# Autodesk Inventor assembly: Trilho 60 min - 12 horas montado
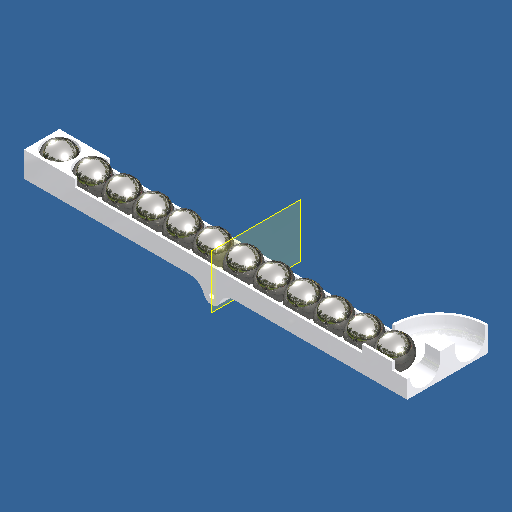
[picture p0: Inventor's stored thumbnail of the model, 512x512]
Saved by Autodesk Inventor 2024 (Build 280153000, 153)
## iProperties
Created: 2023-05-16
Part Number: Trilho 60 min - 12 horas montado
Document SubType Name: Assembly
Designer: jpjoa
Mass: 338.261 g
Surface Area: 330.699 cm^2
Volume: 65.9182 cm^3
Density: 5.13152 g/cm^3
Author: jpjoa
## Documents named in this file (3)
- G:\.shortcut-targets-by-id\16j0rtmAzHYi4Hd3siOhaEHA2SaTRFf-m\Marbles - Peças novas\Trilho 60 min - 12 horas montado.iam
- G:\.shortcut-targets-by-id\16j0rtmAzHYi4Hd3siOhaEHA2SaTRFf-m\Marbles - Peças novas\Trilho 60 min - 12 horas.ipt
- G:\.shortcut-targets-by-id\16j0rtmAzHYi4Hd3siOhaEHA2SaTRFf-m\Marbles - Peças novas\Bola.ipt
## Components (13 placed, 2 different names)
1. Trilho 60 min - 12 horas:1 — Coincidente:1, Coincidente:2, Coincidente:3, Coincidente:4, Coincidente:5, Coincidente:6, Coincidente:7, Coincidente:8, Coincidente:9, Coincidente:10, Coincidente:11, Coincidente:12
2. Bola:1 — Coincidente:1
3. Bola:2 — Coincidente:2, Tangente:1
4. Bola:3 — Coincidente:3, Tangente:1, Tangente:2
5. Bola:4 — Coincidente:4, Tangente:2, Tangente:3
6. Bola:5 — Coincidente:5, Tangente:3, Tangente:4
7. Bola:6 — Coincidente:6, Tangente:4, Tangente:5
8. Bola:7 — Coincidente:7, Tangente:5, Tangente:6
9. Bola:8 — Coincidente:8, Tangente:6, Tangente:7
10. Bola:9 — Coincidente:9, Tangente:7, Tangente:8
11. Bola:10 — Coincidente:10, Tangente:8, Tangente:9
12. Bola:11 — Coincidente:11, Tangente:9, Tangente:10
13. Bola:12 — Coincidente:12, Tangente:10
## Relationships (22: Mate 12, Tangent 10)
- Coincidente:1 [Mate]: Trilho 60 min - 12 horas:1 ↔ Bola:1
- Coincidente:2 [Mate]: Trilho 60 min - 12 horas:1 ↔ Bola:2
- Coincidente:3 [Mate]: Trilho 60 min - 12 horas:1 ↔ Bola:3
- Coincidente:4 [Mate]: Trilho 60 min - 12 horas:1 ↔ Bola:4
- Coincidente:5 [Mate]: Trilho 60 min - 12 horas:1 ↔ Bola:5
- Coincidente:6 [Mate]: Trilho 60 min - 12 horas:1 ↔ Bola:6
- Coincidente:7 [Mate]: Trilho 60 min - 12 horas:1 ↔ Bola:7
- Coincidente:8 [Mate]: Trilho 60 min - 12 horas:1 ↔ Bola:8
- Coincidente:9 [Mate]: Trilho 60 min - 12 horas:1 ↔ Bola:9
- Coincidente:10 [Mate]: Trilho 60 min - 12 horas:1 ↔ Bola:10
- Coincidente:11 [Mate]: Trilho 60 min - 12 horas:1 ↔ Bola:11
- Tangente:1: Bola:2 ↔ Bola:3
- Tangente:2: Bola:3 ↔ Bola:4
- Tangente:3: Bola:4 ↔ Bola:5
- Tangente:4: Bola:5 ↔ Bola:6
- Tangente:5: Bola:6 ↔ Bola:7
- Tangente:6: Bola:7 ↔ Bola:8
- Tangente:7: Bola:8 ↔ Bola:9
- Tangente:8: Bola:9 ↔ Bola:10
- Tangente:9: Bola:10 ↔ Bola:11
- Coincidente:12 [Mate]: Trilho 60 min - 12 horas:1 ↔ Bola:12
- Tangente:10: Bola:11 ↔ Bola:12
